# Autodesk Inventor assembly: ShooterIdea2
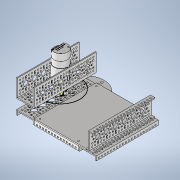
[picture p0: Inventor's stored thumbnail of the model, 180x180]
Saved by Autodesk Inventor 2021 (Build 250183000, 183)
## iProperties
Created: 2021-02-26
Part Number: ShooterIdea2
Document SubType Name: Assembly
Designer: deli
Sending System: Autodesk Inventor 2021
Preprocessor: ST-DEVELOPER v18.1
Title: C:\Users\gfellows\Downloads\ShooterIdea2.stp
Author: gfellows
## Documents named in this file (15)
- C:\Users\deli\OneDrive - Eastside Preparatory School\FTC\Ultamite Goal\Cad\8103-CAD\ShooterIdea2.iam
- C:\Users\deli\OneDrive - Eastside Preparatory School\FTC\Ultamite Goal\Cad\8103-CAD\5000-0002-4008.ipt
- C:\Users\deli\OneDrive - Eastside Preparatory School\FTC\Ultamite Goal\Cad\8103-CAD\1311-0016-4008 assembly.ipt
- C:\Users\deli\OneDrive - Eastside Preparatory School\FTC\Ultamite Goal\Cad\8103-CAD\1611-0514-4008.ipt
- C:\Users\deli\OneDrive - Eastside Preparatory School\FTC\Ultamite Goal\Cad\8103-CAD\1613-0516-0008 assembly with 16mm OD washers.ipt
- C:\Users\deli\OneDrive - Eastside Preparatory School\FTC\Ultamite Goal\Cad\8103-CAD\1121-0006-0168.ipt
- C:\Users\deli\OneDrive - Eastside Preparatory School\FTC\Ultamite Goal\Cad\8103-CAD\2802-0004-0008.ipt
- C:\Users\deli\OneDrive - Eastside Preparatory School\FTC\Ultamite Goal\Cad\8103-CAD\90657A113_ZINC-PLATED STEEL NARROW CHEESE HEAD SLOTTED SCREW.ipt
- C:\Users\deli\OneDrive - Eastside Preparatory School\FTC\Ultamite Goal\Cad\8103-CAD\1121-0004-0120.ipt
- C:\Users\deli\OneDrive - Eastside Preparatory School\FTC\Ultamite Goal\Cad\8103-CAD\bottom plate.ipt
- C:\Users\deli\OneDrive - Eastside Preparatory School\FTC\Ultamite Goal\Cad\8103-CAD\1205-0001-0003.ipt
- C:\Users\deli\OneDrive - Eastside Preparatory School\FTC\Ultamite Goal\Cad\8103-CAD\1205-0001-0003_MIR.ipt
- C:\Users\deli\OneDrive - Eastside Preparatory School\FTC\Ultamite Goal\Cad\8103-CAD\wheel.ipt
- C:\Users\deli\OneDrive - Eastside Preparatory School\FTC\Ultamite Goal\Cad\8103-CAD\ShooterWheel.ipt
- C:\Users\deli\OneDrive - Eastside Preparatory School\FTC\Ultamite Goal\Cad\8103-CAD\1120-0006-0168.ipt
## Components (25 placed, 14 different names)
1. 5000-0002-4008:1 — Mate:8, Mate:12
2. 1311-0016-4008 assembly:1
3. 1611-0514-4008:1
4. 1613-0516-0008 assembly with 16mm OD washers:1
5. 1121-0006-0168:1 — Flush:1, Flush:2, Mate:9, Mate:11, Flush:3, Flush:7, Mate:13, Mate:14, Mate:15, Mate:16, Flush:8, Flush:9, Mate:20, Mate:21
6. 2802-0004-0008:1
7. 2802-0004-0008:6
8. 2802-0004-0008:7
9. 2802-0004-0008:8
10. 90657A113_ZINC-PLATED STEEL NARROW CHEESE HEAD SLOTTED SCREW:1
11. 90657A113_ZINC-PLATED STEEL NARROW CHEESE HEAD SLOTTED SCREW:2
12. 90657A113_ZINC-PLATED STEEL NARROW CHEESE HEAD SLOTTED SCREW:3
13. 90657A113_ZINC-PLATED STEEL NARROW CHEESE HEAD SLOTTED SCREW:4
14. 1121-0006-0168:3 — Flush:5, Flush:6, Flush:10, Flush:11, Mate:17, Mate:18, Mate:23, Mate:24, Mate:25
15. 1121-0004-0120:1 — Mate:11, Flush:3, Flush:4, Flush:5, Flush:7, Flush:10, Flush:11, Mate:17, Mate:19, Mate:22
16. 1121-0004-0120:2 — Mate:16, Flush:8, Flush:9
17. bottom plate:1 — Flush:4, Mate:18, Mate:22
18. 1205-0001-0003:1 — Mate:19, Mate:20, Mate:21
19. 1205-0001-0003:2 — Mate:13, Mate:14, Mate:15
20. 1205-0001-0003_MIR:1
21. 1205-0001-0003_MIR:2
22. 1121-0006-0168:4 — Flush:6, Mate:23, Mate:24, Mate:25
23. wheel:2
24. ShooterWheel:1 — Mate:10, Mate:12
25. 1120-0006-0168:1 — Mate:8, Flush:1, Flush:2, Mate:9, Mate:10
## Relationships (29: Mate 18, Flush 11)
- Mate:8: 5000-0002-4008:1 ↔ 1120-0006-0168:1
- Flush:1: 1121-0006-0168:1 ↔ 1120-0006-0168:1
- Flush:2: 1121-0006-0168:1 ↔ 1120-0006-0168:1
- Mate:9 (27 mm): 1121-0006-0168:1 ↔ 1120-0006-0168:1
- Mate:10: ShooterWheel:1 ↔ 1120-0006-0168:1
- Mate:11: 1121-0006-0168:1 ↔ 1121-0004-0120:1
- Flush:3: 1121-0006-0168:1 ↔ 1121-0004-0120:1
- Flush:4: 1121-0004-0120:1 ↔ bottom plate:1
- Flush:5: 1121-0006-0168:3 ↔ 1121-0004-0120:1
- Flush:6: 1121-0006-0168:3 ↔ 1121-0006-0168:4
- Mate:12: 5000-0002-4008:1 ↔ ShooterWheel:1
- Flush:7: 1121-0006-0168:1 ↔ 1121-0004-0120:1
- Mate:13: 1121-0006-0168:1 ↔ 1205-0001-0003:2
- Mate:14: 1121-0006-0168:1 ↔ 1205-0001-0003:2
- Mate:15: 1121-0006-0168:1 ↔ 1205-0001-0003:2
- Mate:16: 1121-0006-0168:1 ↔ 1121-0004-0120:2
- Flush:8: 1121-0006-0168:1 ↔ 1121-0004-0120:2
- Flush:9: 1121-0006-0168:1 ↔ 1121-0004-0120:2
- Flush:10: 1121-0006-0168:3 ↔ 1121-0004-0120:1
- Flush:11: 1121-0006-0168:3 ↔ 1121-0004-0120:1
- Mate:17: 1121-0006-0168:3 ↔ 1121-0004-0120:1
- Mate:18: 1121-0006-0168:3 ↔ bottom plate:1
- Mate:19: 1121-0004-0120:1 ↔ 1205-0001-0003:1
- Mate:20: 1121-0006-0168:1 ↔ 1205-0001-0003:1
- Mate:21: 1121-0006-0168:1 ↔ 1205-0001-0003:1
- Mate:22: 1121-0004-0120:1 ↔ bottom plate:1
- Mate:23: 1121-0006-0168:3 ↔ 1121-0006-0168:4
- Mate:24: 1121-0006-0168:3 ↔ 1121-0006-0168:4
- Mate:25: 1121-0006-0168:3 ↔ 1121-0006-0168:4
